# Autodesk Inventor assembly: Roof Extension Assembly
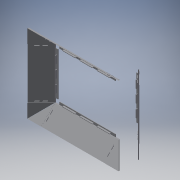
[picture p0: Inventor's stored thumbnail of the model, 180x180]
Saved by Autodesk Inventor 2017 (Build 210142000, 142)
## iProperties
Created: 2018-03-30
Part Number: Roof Extension Assembly
Document SubType Name: Assembly
Designer: Arjuna
Author: Arjuna
## Documents named in this file (6)
- D:\Users\Arjuna\Documents\NTU\FYP\Hardware\Roof Extension Assembly.iam
- D:\Users\Arjuna\Documents\NTU\FYP\Hardware\Roof Width Extension.ipt
- D:\Users\Arjuna\Documents\NTU\FYP\Hardware\Roof Length Extension.ipt
- D:\Users\Arjuna\Documents\NTU\FYP\Hardware\Top Roof.ipt
- D:\Users\Arjuna\Documents\NTU\FYP\Hardware\Roof Extension Right Attachment.ipt
- D:\Users\Arjuna\Documents\NTU\FYP\Hardware\Roof Extension Left Attachment.ipt
## Components (13 placed, 5 different names)
1. Roof Width Extension:1 — Mate:10, Mate:14, Mate:23, Mate:24, Flush:4, Flush:10, Mate:32, Mate:33, Flush:13
2. Roof Width Extension:2 — Mate:12, Mate:16, Mate:19, Mate:20, Flush:6, Mate:26, Mate:28, Mate:29, Flush:15
3. Roof Length Extension:1 — Mate:11, Mate:13, Mate:21, Mate:22, Flush:7, Mate:27, Mate:30, Mate:31, Flush:12
4. Roof Length Extension:2 — Mate:9, Mate:15, Mate:17, Mate:18, Flush:5, Flush:11, Mate:34, Mate:35, Flush:14
5. Top Roof:1 — Mate:9, Mate:10, Mate:11, Mate:12, Mate:13, Mate:14, Mate:15, Mate:16, Mate:25, Flush:8, Flush:9, Mate:26, Flush:10, Mate:27, Flush:11
6. Roof Extension Right Attachment:1 — Mate:21, Mate:22, Flush:7
7. Roof Extension Right Attachment:2 — Mate:19, Mate:20, Flush:6
8. Roof Extension Right Attachment:3 — Mate:17, Mate:18, Flush:5
9. Roof Extension Right Attachment:4 — Mate:23, Mate:24, Flush:4
10. Roof Extension Left Attachment:1 — Mate:32, Mate:33, Flush:13
11. Roof Extension Left Attachment:2 — Mate:30, Mate:31, Flush:12
12. Roof Extension Left Attachment:3 — Mate:34, Mate:35, Flush:14
13. Roof Extension Left Attachment:4 — Mate:28, Mate:29, Flush:15
## Relationships (39: Mate 27, Flush 12)
- Mate:9: Roof Length Extension:2 ↔ Top Roof:1
- Mate:10: Roof Width Extension:1 ↔ Top Roof:1
- Mate:11: Roof Length Extension:1 ↔ Top Roof:1
- Mate:12 (75 mm): Roof Width Extension:2 ↔ Top Roof:1
- Mate:13: Roof Length Extension:1 ↔ Top Roof:1
- Mate:14: Roof Width Extension:1 ↔ Top Roof:1
- Mate:15: Roof Length Extension:2 ↔ Top Roof:1
- Mate:16: Roof Width Extension:2 ↔ Top Roof:1
- Mate:17: Roof Length Extension:2 ↔ Roof Extension Right Attachment:3
- Mate:18: Roof Length Extension:2 ↔ Roof Extension Right Attachment:3
- Mate:19: Roof Width Extension:2 ↔ Roof Extension Right Attachment:2
- Mate:20: Roof Width Extension:2 ↔ Roof Extension Right Attachment:2
- Mate:21: Roof Length Extension:1 ↔ Roof Extension Right Attachment:1
- Mate:22: Roof Length Extension:1 ↔ Roof Extension Right Attachment:1
- Mate:23: Roof Width Extension:1 ↔ Roof Extension Right Attachment:4
- Mate:24: Roof Width Extension:1 ↔ Roof Extension Right Attachment:4
- Flush:4: Roof Width Extension:1 ↔ Roof Extension Right Attachment:4
- Flush:5: Roof Length Extension:2 ↔ Roof Extension Right Attachment:3
- Flush:6: Roof Width Extension:2 ↔ Roof Extension Right Attachment:2
- Flush:7: Roof Length Extension:1 ↔ Roof Extension Right Attachment:1
- Mate:25: Top Roof:1
- Flush:8: Top Roof:1
- Flush:9: Top Roof:1
- Mate:26: Roof Width Extension:2 ↔ Top Roof:1
- Flush:10: Roof Width Extension:1 ↔ Top Roof:1
- Mate:27: Roof Length Extension:1 ↔ Top Roof:1
- Flush:11: Roof Length Extension:2 ↔ Top Roof:1
- Mate:28: Roof Width Extension:2 ↔ Roof Extension Left Attachment:4
- Mate:29: Roof Width Extension:2 ↔ Roof Extension Left Attachment:4
- Mate:30: Roof Length Extension:1 ↔ Roof Extension Left Attachment:2
- Mate:31: Roof Length Extension:1 ↔ Roof Extension Left Attachment:2
- Mate:32: Roof Width Extension:1 ↔ Roof Extension Left Attachment:1
- Mate:33: Roof Width Extension:1 ↔ Roof Extension Left Attachment:1
- Mate:34: Roof Length Extension:2 ↔ Roof Extension Left Attachment:3
- Mate:35: Roof Length Extension:2 ↔ Roof Extension Left Attachment:3
- Flush:12: Roof Length Extension:1 ↔ Roof Extension Left Attachment:2
- Flush:13: Roof Width Extension:1 ↔ Roof Extension Left Attachment:1
- Flush:14: Roof Length Extension:2 ↔ Roof Extension Left Attachment:3
- Flush:15: Roof Width Extension:2 ↔ Roof Extension Left Attachment:4
